# Autodesk Inventor assembly: forkMountForDecTripV01
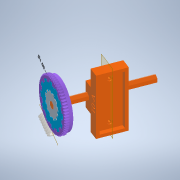
[picture p0: Inventor's stored thumbnail of the model, 180x180]
Saved by Autodesk Inventor 2021.1 (Build 251245010, 245A)
## iProperties
Created: 2020-11-06
Part Number: forkMountForDecTripV01
Document SubType Name: Assembly
Designer: robst
Author: robst
## Documents named in this file (9)
- C:\git\CAD-Development\robSteele\ShapeWays\TelescopeProjects\TelescopeMount\forkMountForDecTripV01.iam
- C:\git\CAD-Development\robSteele\ShapeWays\TelescopeProjects\TelescopeMount\telescopeTube.ipt
- C:\git\CAD-Development\robSteele\ShapeWays\TelescopeProjects\TelescopeMount\celestronTubeBracket.ipt
- C:\git\CAD-Development\robSteele\ShapeWays\TelescopeProjects\TelescopeMount\triangleSupportForMount.ipt
- C:\git\CAD-Development\robSteele\ShapeWays\TelescopeProjects\TelescopeMount\tripod.ipt
- C:\git\CAD-Development\robSteele\ShapeWays\TelescopeProjects\TelescopeMount\forkMountForDecTripV01\Design Accelerator\Worm Gears5.iam
- C:\git\CAD-Development\robSteele\ShapeWays\TelescopeProjects\TelescopeMount\connectorToTubeBracketWithOffsetHexShaft-V01.ipt
- C:\git\CAD-Development\robSteele\ShapeWays\TelescopeProjects\TelescopeMount\SplineLock\outerPartOfLock.ipt
- C:\git\CAD-Development\robSteele\ShapeWays\TelescopeProjects\TelescopeMount\SplineLock\centerPartOfLock.ipt
## Components (9 placed, 8 different names)
1. telescopeTube:1 — Insert:1, Flush:1
2. connectorToTubeBracketWithOffsetHexShaft-V01:1 — Mate:10, Mate:11, Mate:12, Mate:13, Mate:14, Mate:15, Flush:3, Flush:4, Mate:16, Mate:17
3. celestronTubeBracket:1 — Insert:1, Mate:13, Mate:14, Mate:15
4. celestronTubeBracket:2 — Mate:10, Mate:11, Mate:12
5. triangleSupportForMount:1 — Mate:7, Mate:8, Angle:1
6. tripod:1 — Mate:7, Mate:8, Flush:1
7. Worm Gears:1 [sub-assembly] — Insert:2, Angle:1, Flush:5
8. outerPartOfLock:1 — Insert:3, Flush:5
9. centerPartOfLock:1 — Flush:3, Flush:4, Mate:16, Mate:17, Insert:2, Insert:3
## Relationships (18: Mate 10, Flush 4, Insert 3, Angle 1)
- Insert:1 (149.225 mm): telescopeTube:1 ↔ celestronTubeBracket:1
- Mate:7: triangleSupportForMount:1 ↔ tripod:1
- Mate:8: triangleSupportForMount:1 ↔ tripod:1
- Flush:1: telescopeTube:1 ↔ tripod:1
- Mate:10: connectorToTubeBracketWithOffsetHexShaft-V01:1 ↔ celestronTubeBracket:2
- Mate:11: connectorToTubeBracketWithOffsetHexShaft-V01:1 ↔ celestronTubeBracket:2
- Mate:12: connectorToTubeBracketWithOffsetHexShaft-V01:1 ↔ celestronTubeBracket:2
- Mate:13: connectorToTubeBracketWithOffsetHexShaft-V01:1 ↔ celestronTubeBracket:1
- Mate:14: connectorToTubeBracketWithOffsetHexShaft-V01:1 ↔ celestronTubeBracket:1
- Mate:15: connectorToTubeBracketWithOffsetHexShaft-V01:1 ↔ celestronTubeBracket:1
- Flush:3: connectorToTubeBracketWithOffsetHexShaft-V01:1 ↔ centerPartOfLock:1
- Flush:4: connectorToTubeBracketWithOffsetHexShaft-V01:1 ↔ centerPartOfLock:1
- Mate:16: connectorToTubeBracketWithOffsetHexShaft-V01:1 ↔ centerPartOfLock:1
- Mate:17: connectorToTubeBracketWithOffsetHexShaft-V01:1 ↔ centerPartOfLock:1
- Insert:2: Worm Gears:1 ↔ centerPartOfLock:1
- Angle:1 (0 deg): triangleSupportForMount:1 ↔ Worm Gears:1
- Insert:3: outerPartOfLock:1 ↔ centerPartOfLock:1
- Flush:5: Worm Gears:1 ↔ outerPartOfLock:1
